# Autodesk Inventor assembly: servo_top_with_nuts
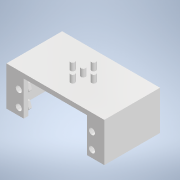
[picture p0: Inventor's stored thumbnail of the model, 180x180]
Saved by Autodesk Inventor 2021.4 (Build 254397000, 397)
## iProperties
Created: 2022-07-26
Part Number: servo_top_with_nuts
Document SubType Name: Assembly
Designer: isamu
Author: isamu
## Documents named in this file (5)
- D:\personal_projects\robot\inventor\2021_matlab_compat _v2\servo_top_with_nuts.iam
- D:\personal_projects\robot\exports\frames\servo frame with top.ipt
- D:\personal_projects\robot\exports\screws\m3x8.ipt
- D:\personal_projects\robot\exports\screws\m4x12.ipt
- D:\personal_projects\robot\exports\screws\m4 nuts.ipt
## Components (12 placed, 4 different names)
1. servo frame with top:1 — Insert:1, Insert:2, Insert:3, Insert:4, Insert:5, Insert:6, Insert:7, Insert:8, Insert:9, Insert:10, Insert:11
2. m3x8:1 — Insert:5
3. m3x8:2 — Insert:4
4. m3x8:3 — Insert:3
5. m3x8:4 — Insert:1
6. m3x8:5 — Insert:2
7. m4x12:1 — Insert:7
8. m4 nuts:1 — Insert:6
9. m4 nuts:2 — Insert:9
10. m4 nuts:3 — Insert:10
11. m4 nuts:4 — Insert:11
12. m4 nuts:5 — Insert:8
## Relationships (11: Insert 11)
- Insert:1: servo frame with top:1 ↔ m3x8:4
- Insert:2: servo frame with top:1 ↔ m3x8:5
- Insert:3: servo frame with top:1 ↔ m3x8:3
- Insert:4: servo frame with top:1 ↔ m3x8:2
- Insert:5: servo frame with top:1 ↔ m3x8:1
- Insert:6: servo frame with top:1 ↔ m4 nuts:1
- Insert:7: servo frame with top:1 ↔ m4x12:1
- Insert:8: servo frame with top:1 ↔ m4 nuts:5
- Insert:9: servo frame with top:1 ↔ m4 nuts:2
- Insert:10: servo frame with top:1 ↔ m4 nuts:3
- Insert:11: servo frame with top:1 ↔ m4 nuts:4
